# Autodesk Inventor assembly: Naroznik v2
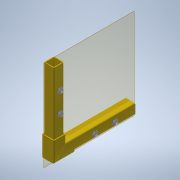
[picture p0: Inventor's stored thumbnail of the model, 180x180]
Saved by Autodesk Inventor 2021 (Build 250183000, 183)
## iProperties
Created: 2024-04-18
Part Number: Naroznik v2
Document SubType Name: Assembly
Designer: Michal
Author: Michal
## Documents named in this file (5)
- C:\Users\Michal\Documents\GitHub\PNW_PhotoBoothFrame_3D\Naroznik v2.iam
- C:\Users\Michal\Documents\GitHub\PNW_PhotoBoothFrame_3D\M8x15.ipt
- C:\Users\Michal\Documents\GitHub\PNW_PhotoBoothFrame_3D\Naroznik v2  profil 1.ipt
- C:\Users\Michal\Documents\GitHub\PNW_PhotoBoothFrame_3D\Naroznik v2 profil 2.ipt
- C:\Users\Michal\Documents\GitHub\PNW_PhotoBoothFrame_3D\Naroznik v2 profil 4.ipt
## Components (8 placed, 4 different names)
1. Naroznik v2 profil 2:1 — Mate:1, Flush:1, Mate:2, Mate:3, Mate:4, Mate:7, Flush:11, Mate:10
2. Naroznik v2  profil 1:1 — Mate:1, Flush:1, Mate:2, Mate:5, Mate:6, Flush:6
3. M8x15:1 — Mate:3, Flush:2, Flush:3, Flush:4, Mate:7
4. M8x15:2 — Mate:4, Flush:2
5. M8x15:3 — Mate:5, Flush:3
6. M8x15:4 — Mate:6, Flush:4
7. Naroznik v2 profil 4:1 — Mate:8, Flush:5, Mate:9, Mate:10
8. Naroznik v2 profil 4:2 — Mate:8, Flush:5, Mate:9, Flush:11, Flush:6
## Relationships (17: Mate 10, Flush 7)
- Mate:1: Naroznik v2 profil 2:1 ↔ Naroznik v2  profil 1:1
- Flush:1: Naroznik v2 profil 2:1 ↔ Naroznik v2  profil 1:1
- Mate:2: Naroznik v2 profil 2:1 ↔ Naroznik v2  profil 1:1
- Mate:3: Naroznik v2 profil 2:1 ↔ M8x15:1
- Mate:4: Naroznik v2 profil 2:1 ↔ M8x15:2
- Mate:5: Naroznik v2  profil 1:1 ↔ M8x15:3
- Mate:6: Naroznik v2  profil 1:1 ↔ M8x15:4
- Flush:2: M8x15:1 ↔ M8x15:2
- Flush:3: M8x15:1 ↔ M8x15:3
- Flush:4: M8x15:1 ↔ M8x15:4
- Mate:7 (3 mm): Naroznik v2 profil 2:1 ↔ M8x15:1
- Mate:8: Naroznik v2 profil 4:1 ↔ Naroznik v2 profil 4:2
- Flush:5: Naroznik v2 profil 4:1 ↔ Naroznik v2 profil 4:2
- Mate:9: Naroznik v2 profil 4:1 ↔ Naroznik v2 profil 4:2
- Flush:11: Naroznik v2 profil 2:1 ↔ Naroznik v2 profil 4:2
- Flush:6: Naroznik v2  profil 1:1 ↔ Naroznik v2 profil 4:2
- Mate:10: Naroznik v2 profil 2:1 ↔ Naroznik v2 profil 4:1
